# Autodesk Inventor assembly: Übertragung des Zahnriemens
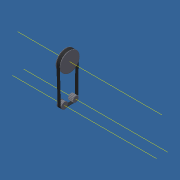
[picture p0: Inventor's stored thumbnail of the model, 180x180]
Saved by Autodesk Inventor 2016 (Build 200138000, 138)
## iProperties
Created: 2015-08-25
Part Number: Übertragung des Zahnriemens
Document SubType Name: Assembly
Designer: 4ndreas
Mass: 93.7371 g
Surface Area: 87.8411 cm^2
Volume: 12.7185 cm^3
Density: 7.37011 g/cm^3
ClientObjectVersion: 1
Author: 4ndreas
## Documents named in this file (5)
- C:\Users\4ndreas\Documents\Inventor\RobotARM v2\v4\Wrist\Konstruktions-Assistent\Übertragung des Zahnriemens2.iam
- C:\Users\4ndreas\Documents\Inventor\RobotARM v2\v4\Wrist\Konstruktions-Assistent\Zahnriemen2.ipt
- C:\Users\4ndreas\Documents\Inventor\RobotARM v2\v4\Wrist\Konstruktions-Assistent\Synchrone Riemenscheibe12.ipt
- C:\Users\4ndreas\Documents\Inventor\RobotARM v2\v4\Wrist\Konstruktions-Assistent\Synchrone Riemenscheibe22.ipt
- C:\Users\4ndreas\Documents\Inventor\RobotARM v2\v4\Wrist\Konstruktions-Assistent\Synchrone Riemenscheibe31.ipt
## Components (4 placed, 4 different names)
1. Zahnriemen:1 — Fluchtend:1, Passend:1, Passend:2, Fluchtend:2, Passend:3, Passend:4, Fluchtend:3, Passend:5, Passend:6
2. Synchrone Riemenscheibe1:1 — Fluchtend:1, Passend:1, Passend:2, Drehung:1, Drehung:2
3. Synchrone Riemenscheibe2:1 — Fluchtend:2, Passend:3, Drehung:1, Passend:4
4. Synchrone Riemenscheibe3:1 — Fluchtend:3, Passend:5, Drehung:2, Passend:6
## Relationships (11: Mate 6, Flush 3, RelateRotation 2)
- Fluchtend:1 [Flush]: Zahnriemen:1 ↔ Synchrone Riemenscheibe1:1
- Passend:1 [Mate]: Zahnriemen:1 ↔ Synchrone Riemenscheibe1:1
- Passend:2 [Mate]: Zahnriemen:1 ↔ Synchrone Riemenscheibe1:1
- Fluchtend:2 [Flush]: Zahnriemen:1 ↔ Synchrone Riemenscheibe2:1
- Passend:3 [Mate]: Zahnriemen:1 ↔ Synchrone Riemenscheibe2:1
- Drehung:1 [RelateRotation] (3 ul): Synchrone Riemenscheibe1:1 ↔ Synchrone Riemenscheibe2:1
- Passend:4 [Mate]: Zahnriemen:1 ↔ Synchrone Riemenscheibe2:1
- Fluchtend:3 [Flush]: Zahnriemen:1 ↔ Synchrone Riemenscheibe3:1
- Passend:5 [Mate]: Zahnriemen:1 ↔ Synchrone Riemenscheibe3:1
- Drehung:2 [RelateRotation] (1 ul): Synchrone Riemenscheibe1:1 ↔ Synchrone Riemenscheibe3:1
- Passend:6 [Mate]: Zahnriemen:1 ↔ Synchrone Riemenscheibe3:1
